# Autodesk Inventor assembly: 17032021
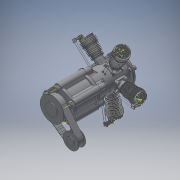
[picture p0: Inventor's stored thumbnail of the model, 180x180]
Saved by Autodesk Inventor 2018 (Build 220112000, 112)
## iProperties
Created: 2021-03-15
Part Number: 17032021
Document SubType Name: Assembly
Designer: Jyoti Soni
Author: Jyoti Soni
## Documents named in this file (3)
- C:\Users\Jyoti Soni\Desktop\asm\15032021\17032021.iam
- C:\Users\Jyoti Soni\Desktop\asm\15032021\cylinder asm.iam
- C:\Users\Jyoti Soni\Desktop\chain sproket.ipt
## Components (2 placed, 2 different names)
1. cylinder asm:1 [sub-assembly] — Mate:5
2. chain sproket:1 — Mate:4, Mate:5
## Relationships (2: Mate 2)
- Mate:4: chain sproket:1
- Mate:5 (10 mm): cylinder asm:1 ↔ chain sproket:1
